# Autodesk Inventor assembly: XY Joint Left
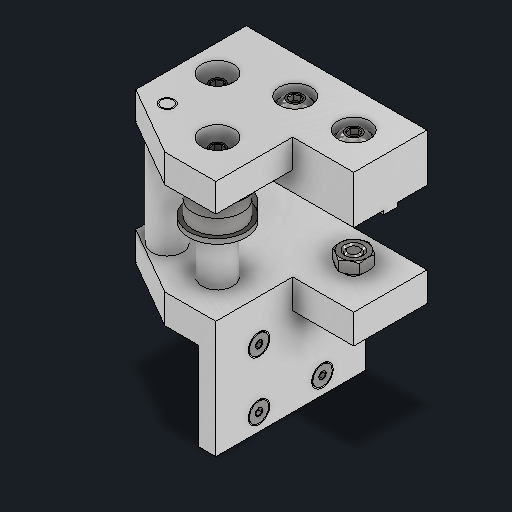
[picture p0: Inventor's stored thumbnail of the model, 512x512]
Saved by Autodesk Inventor 2025.1 (Build 291241020, 241B)
## iProperties
Created: 2025-05-09
Part Number: XY Joint Left
Document SubType Name: Assembly
Designer: AdminForWorker
Title: XY Joint Left
Author: AdminForWorker
## Documents named in this file (10)
- C:\Users\Joshua Eah\Documents\Voron 0.2\CAD\Master Assembly\X Axis\XY Joint Left.iam
- C:\Users\Joshua Eah\Documents\Voron 0.2\CAD\Machined Parts\XY Joints\XY Joint Left\XY Joint Left.iam
- XY Joint Left.iam
- C:\Users\Joshua Eah\Documents\Voron 0.2\CAD\Master Assembly\Hardware\F623 Stack.iam
- C:\Users\Joshua Eah\Documents\Voron 0.2\CAD\Master Assembly\Hardware\M3 Hexnut.ipt
- C:\Users\Joshua Eah\Documents\Voron 0.2\CAD\Master Assembly\Hardware\M3x25 BHCS.ipt
- C:\Users\Joshua Eah\Documents\Voron 0.2\CAD\Master Assembly\Hardware\M2x6 FHCS.ipt
- C:\Users\Joshua Eah\Documents\Voron 0.2\CAD\Master Assembly\Hardware\M3x12 BHCS.ipt
- C:\Users\Joshua Eah\Documents\Voron 0.2\CAD\Master Assembly\Hardware\M3x6 BHCS.ipt
- C:\Users\Joshua Eah\Documents\Voron 0.2\CAD\Master Assembly\Hardware\M3_Washer.ipt
## Components (19 placed, 8 different names)
1. XY Joint Left:1 [sub-assembly] — Insert:2, Insert:3, Insert:4, Insert:5
2. F623 Stack:2 [sub-assembly]
3. F623 Stack:1 [sub-assembly]
4. M3 Hexnut:1
5. M3 Hexnut:2
6. M3 Hexnut:3
7. M3x25 BHCS:1
8. M2x6 FHCS:1 — Insert:4
9. M2x6 FHCS:2 — Insert:2
10. M2x6 FHCS:3 — Insert:5
11. M2x6 FHCS:4 — Insert:3
12. M3x25 BHCS:2
13. M3x12 BHCS:1
14. M3x12 BHCS:2
15. M3x6 BHCS:1
16. M3 Washer (4):5
17. M3 Washer (4):6
18. M3 Washer (4):7
19. M3 Washer (4):8
## Relationships (5: Insert 5)
- [Insert]: XY Joint Left:1 ↔ M3x12 BHCS:1
- Insert:2: XY Joint Left:1 ↔ M2x6 FHCS:2
- Insert:3: XY Joint Left:1 ↔ M2x6 FHCS:4
- Insert:4: XY Joint Left:1 ↔ M2x6 FHCS:1
- Insert:5: XY Joint Left:1 ↔ M2x6 FHCS:3
